# Autodesk Inventor assembly: 1535_top_assembly
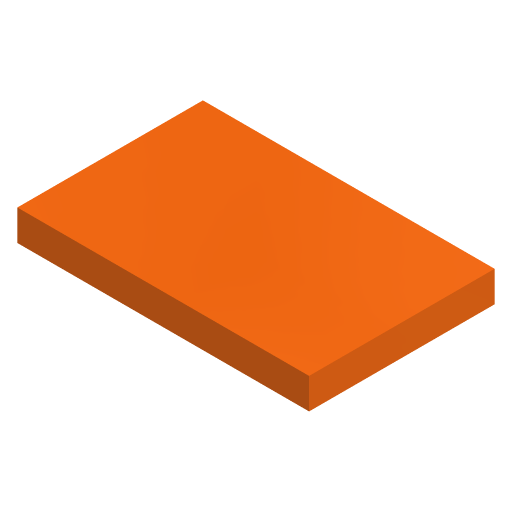
[picture p0: Inventor's stored thumbnail of the model, 512x512]
Saved by Autodesk Inventor 2023 (Build 270158000, 158)
## iProperties
Created: 2024-05-06
Part Number: 1535_top_assembly
Document SubType Name: Assembly
Designer: Thomas
Author: Thomas
## iProperties of the stored document 1535 Top Tub.ipt
Created: 2019-02-13
Part Number: 1535 Top Tub
Material: Generic
Description: STEP AP214
Document SubType Name: Modeling
Designer: Thomas
Density: 1 g/cm^3
Appearance: Default
Sending System: SolidWorks 2016
Preprocessor: SwSTEP 2.0
Title: 1535 Top Tub.STEP
Revision Number: ANY
## iProperties of the stored document 9307K12_Buna-N Rubber Grommets.ipt
Company: Managed by Terraform
Created: 2024-02-22
Part Number: 9307K12_Buna-N Rubber Grommets
Material: Generic
Description: STEP AP203
Document SubType Name: Modeling
Designer: Thomas
Density: 1 g/cm^3
Appearance: Default
Sending System: SolidWorks 2017
Preprocessor: SwSTEP 2.0
Title: 9307K12_Buna-N Rubber Grommets.STEP
Author: Administrator
Revision Number: ANY
## Documents named in this file (8)
- Z:\penguin_1535_radar_case\1535_top_assembly.iam
- **Z:\penguin_1535_radar_case\1535_top_assembly.iam*LocalDocs*xAaaaq1baAaaaaaaaAaaaanm5Bd*1535 Top Tub.ipt
- Z:\penguin_1535_radar_case\lid_panel.ipt
- **Z:\penguin_1535_radar_case\1535_top_assembly.iam*LocalDocs*xAaaaqtcaAaaaaaaaAaaaai12Wb*9307K12_Buna-N Rubber Grommets.ipt
- Z:\penguin_1535_radar_case\lid_tray_mounts\lid_mount_sparkfun_f9p.ipt
- Z:\penguin_1535_radar_case\lid_tray_mounts\backing_nut.ipt
- Z:\penguin_1535_radar_case\reference_cad\1535_step\1535 Top Tub.STEP
- Z:\penguin_1535_radar_case\reference_cad\9307K12_Buna-N Rubber Grommets.STEP
## Components (8 placed, 5 different names)
1. 1535 Top Tub:1 — Insert:5
2. lid_panel:1 — Insert:1, Insert:2, Insert:3, Insert:4, Insert:6, Insert:7, Insert:8, Angle:1
3. 9307K12_Buna-N Rubber Grommets:1 — Insert:1, Insert:5
4. 9307K12_Buna-N Rubber Grommets:2 — Insert:2
5. 9307K12_Buna-N Rubber Grommets:3 — Insert:4
6. 9307K12_Buna-N Rubber Grommets:4 — Insert:3
7. lid_mount_sparkfun_f9p:1 — Insert:6, Insert:7
8. backing_nut:1 — Insert:8, Angle:1
## Relationships (9: Insert 8, Angle 1)
- Insert:1: lid_panel:1 ↔ 9307K12_Buna-N Rubber Grommets:1
- Insert:2: lid_panel:1 ↔ 9307K12_Buna-N Rubber Grommets:2
- Insert:3: lid_panel:1 ↔ 9307K12_Buna-N Rubber Grommets:4
- Insert:4: lid_panel:1 ↔ 9307K12_Buna-N Rubber Grommets:3
- Insert:5: 1535 Top Tub:1 ↔ 9307K12_Buna-N Rubber Grommets:1
- Insert:6: lid_panel:1 ↔ lid_mount_sparkfun_f9p:1
- Insert:7: lid_panel:1 ↔ lid_mount_sparkfun_f9p:1
- Insert:8: lid_panel:1 ↔ backing_nut:1
- Angle:1 (0 deg): lid_panel:1 ↔ backing_nut:1
